# Autodesk Inventor assembly: ForeArmAssembly
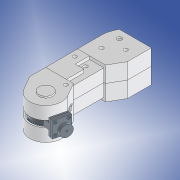
[picture p0: Inventor's stored thumbnail of the model, 180x180]
Saved by Autodesk Inventor 2017 SP1 (Build 210196100, 196)
## iProperties
Created: 2017-06-14
Part Number: ForeArmAssembly
Document SubType Name: Assembly
Designer: zallen
Author: zallen
## Documents named in this file (15)
- C:\Users\Zach\Documents\GitHub\cr-laundry-robot\src\Body\Arm Assembly\Bicep Assembly\BicepAssembly.iam
- C:\Users\Zach\Documents\GitHub\cr-laundry-robot\src\Body\Arm Assembly\Bicep Assembly\BA001.ipt
- C:\Users\Zach\Documents\GitHub\cr-laundry-robot\src\Body\Arm Assembly\Bicep Assembly\BA002.ipt
- C:\Users\Zach\Documents\GitHub\cr-laundry-robot\lib\Stepper Motor - NEMA 17\NEMA17.ipt
- C:\Users\Zach\Documents\GitHub\cr-laundry-robot\src\Body\Arm Assembly\Bicep Assembly\BA003.ipt
- C:\Users\Zach\Documents\GitHub\cr-laundry-robot\src\Body\Arm Assembly\Bicep Assembly\BA004.ipt
- C:\Users\Zach\Documents\GitHub\cr-laundry-robot\src\Body\Arm Assembly\Bicep Assembly\BA005.ipt
- C:\Users\Zach\Documents\GitHub\cr-laundry-robot\src\Body\Arm Assembly\Bicep Assembly\12 x 100mm Shaft.ipt
- C:\Users\Zach\Documents\GitHub\cr-laundry-robot\src\Body\Arm Assembly\Bicep Assembly\BicepAssembly\Design Accelerator\Spur Gears1.iam
- C:\Users\Zach\Documents\GitHub\cr-laundry-robot\lib\6201RS\6201RS.ipt
- C:\Users\Zach\Documents\GitHub\cr-laundry-robot\src\Body\Arm Assembly\Bicep Assembly\BA007.ipt
- C:\Users\Zach\Documents\GitHub\cr-laundry-robot\src\Body\Arm Assembly\Bicep Assembly\BA008.ipt
- C:\Users\Zach\Documents\GitHub\cr-laundry-robot\src\Body\Arm Assembly\Bicep Assembly\BA011.ipt
- C:\Users\Zach\Documents\GitHub\cr-laundry-robot\src\Body\Arm Assembly\Bicep Assembly\BA010.ipt
- C:\Users\Zach\Documents\GitHub\cr-laundry-robot\src\Body\Arm Assembly\Bicep Assembly\10 x  80mm Shaft.ipt
## Components (16 placed, 14 different names)
1. BA001:1 — Mate:1, Mate:4, Mate:8, Mate:12, Mate:52, Mate:54, Mate:55, Mate:56
2. BA002:1 — Mate:1, Mate:4, Mate:53, Mate:57
3. BA003:1 — Mate:8, Mate:12, Mate:16, Mate:17, Mate:58, Mate:59, Mate:60, Mate:62, Mate:63, Mate:64, Mate:65
4. BA004:1 — Mate:44
5. BA005:1 — Mate:16, Mate:17, Mate:19, Mate:20, Mate:38, Mate:66, Mate:67, Mate:68, Mate:69
6. 12 x 100mm Shaft:1 — Mate:19, Mate:20, Mate:35, Mate:44, Mate:46
7. Spur Gears:1 [sub-assembly] — Mate:35, Mate:36, Mate:37, Mate:38, Mate:47, Mate:48, Mate:49, Mate:50, Flush:1, Rotation:1, Mate:66, Mate:67
8. 6201RS:1 — Mate:36, Mate:37
9. 6201RS:2 — Mate:46, Mate:47
10. BA007:1 — Mate:48, Mate:49, Mate:50
11. BA008:1 — Mate:52, Mate:53, Mate:54
12. BA008:2 — Mate:55, Mate:56, Mate:57
13. NEMA17:2 — Mate:58, Mate:59, Mate:60, Mate:61
14. BA011:1 — Mate:61, Flush:1, Rotation:1
15. BA010:1 — Mate:62, Mate:63, Mate:64, Mate:65
16. 10 x  80mm Shaft:1 — Mate:68, Mate:69
## Relationships (38: Mate 36, Flush 1, RelateRotation 1)
- Mate:1: BA001:1 ↔ BA002:1
- Mate:4: BA001:1 ↔ BA002:1
- Mate:8: BA001:1 ↔ BA003:1
- Mate:12: BA001:1 ↔ BA003:1
- Mate:16: BA003:1 ↔ BA005:1
- Mate:17: BA003:1 ↔ BA005:1
- Mate:19: BA005:1 ↔ 12 x 100mm Shaft:1
- Mate:20: BA005:1 ↔ 12 x 100mm Shaft:1
- Mate:35: 12 x 100mm Shaft:1 ↔ Spur Gears:1
- Mate:36: Spur Gears:1 ↔ 6201RS:1
- Mate:37: Spur Gears:1 ↔ 6201RS:1
- Mate:38: BA005:1 ↔ Spur Gears:1
- Mate:44: BA004:1 ↔ 12 x 100mm Shaft:1
- Mate:46: 12 x 100mm Shaft:1 ↔ 6201RS:2
- Mate:47: Spur Gears:1 ↔ 6201RS:2
- Mate:48: Spur Gears:1 ↔ BA007:1
- Mate:49: Spur Gears:1 ↔ BA007:1
- Mate:50: Spur Gears:1 ↔ BA007:1
- Mate:52: BA001:1 ↔ BA008:1
- Mate:53: BA002:1 ↔ BA008:1
- Mate:54: BA001:1 ↔ BA008:1
- Mate:55: BA001:1 ↔ BA008:2
- Mate:56: BA001:1 ↔ BA008:2
- Mate:57: BA002:1 ↔ BA008:2
- Mate:58: BA003:1 ↔ NEMA17:2
- Mate:59: BA003:1 ↔ NEMA17:2
- Mate:60: BA003:1 ↔ NEMA17:2
- Mate:61: NEMA17:2 ↔ BA011:1
- Flush:1: Spur Gears:1 ↔ BA011:1
- Rotation:1 [RelateRotation] (0.7857 ul): Spur Gears:1 ↔ BA011:1
- Mate:62: BA003:1 ↔ BA010:1
- Mate:63: BA003:1 ↔ BA010:1
- Mate:64: BA003:1 ↔ BA010:1
- Mate:65: BA003:1 ↔ BA010:1
- Mate:66: BA005:1 ↔ Spur Gears:1
- Mate:67: BA005:1 ↔ Spur Gears:1
- Mate:68: BA005:1 ↔ 10 x  80mm Shaft:1
- Mate:69: BA005:1 ↔ 10 x  80mm Shaft:1
